# Autodesk Inventor assembly: Base
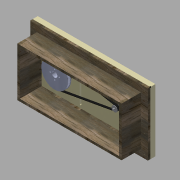
[picture p0: Inventor's stored thumbnail of the model, 180x180]
Saved by Autodesk Inventor 2019 (Build 230136000, 136)
## iProperties
Created: 2021-11-07
Part Number: Base
Document SubType Name: Assembly
Designer: Mohamed
Author: Mohamed
## Documents named in this file (11)
- F:\Semester 7\Design of mechatronics 1\SSCARA Robot\Base.iam
- F:\Semester 7\Design of mechatronics 1\SSCARA Robot\b_base_support 3.ipt
- F:\Semester 7\Design of mechatronics 1\SSCARA Robot\b_base_support 2.ipt
- F:\Semester 7\Design of mechatronics 1\SSCARA Robot\b_Base_support 1.ipt
- F:\Semester 7\Design of mechatronics 1\SSCARA Robot\thrust bearing_40mm.iam
- F:\Semester 7\Design of mechatronics 1\SSCARA Robot\b_base_cover_1.ipt
- F:\Semester 7\Design of mechatronics 1\SSCARA Robot\110 teeth gt2 pulley.ipt
- F:\Semester 7\Design of mechatronics 1\SSCARA Robot\nema 17 motor.ipt
- F:\Semester 7\Design of mechatronics 1\SSCARA Robot\ball bearing 35mm.ipt
- F:\Semester 7\Design of mechatronics 1\SSCARA Robot\GT2 pulley 20 teeth.ipt
- F:\Semester 7\Design of mechatronics 1\SSCARA Robot\belt_460mm.ipt
## Components (13 placed, 10 different names)
1. b_base_support 3:1 — Mate:4, Flush:1, Flush:2
2. b_base_support 2:1 — Mate:6, Flush:5, Flush:6
3. b_Base_support 1:1 — Mate:1, Mate:2, Mate:3, Mate:4, Flush:1, Mate:5, Flush:3, Mate:6, Flush:6, Mate:19, Flush:8, Flush:9
4. b_base_support 3:2 — Mate:5, Flush:3, Flush:4, Flush:5
5. b_base_support 2:2 — Mate:1, Mate:2, Mate:3, Flush:2, Flush:4
6. thrust bearing_40mm:1 [sub-assembly] — Mate:7, Mate:8, Mate:12
7. thrust bearing_40mm:2 [sub-assembly] — Mate:13, Mate:14
8. b_base_cover_1:1 — Mate:9, Mate:10, Mate:12, Mate:13, Mate:15, Mate:16, Mate:17, Mate:19, Flush:8, Flush:9
9. 110 teeth gt2 pulley:1 — Mate:7, Mate:8, Mate:11, Mate:14, Flush:7, Mate:21
10. nema 17 motor:1 — Mate:15, Mate:16, Mate:17, Mate:18
11. ball bearing 35mm:1 — Mate:9, Mate:10, Mate:11
12. GT2 pulley 20 teeth:1 — Mate:18, Flush:7, Mate:20, Mate:22
13. belt_460mm:1 — Mate:20, Mate:21, Mate:22
## Relationships (31: Mate 22, Flush 9)
- Mate:1: b_Base_support 1:1 ↔ b_base_support 2:2
- Mate:2: b_Base_support 1:1 ↔ b_base_support 2:2
- Mate:3: b_Base_support 1:1 ↔ b_base_support 2:2
- Mate:4: b_base_support 3:1 ↔ b_Base_support 1:1
- Flush:1: b_base_support 3:1 ↔ b_Base_support 1:1
- Flush:2: b_base_support 3:1 ↔ b_base_support 2:2
- Mate:5: b_Base_support 1:1 ↔ b_base_support 3:2
- Flush:3: b_Base_support 1:1 ↔ b_base_support 3:2
- Flush:4: b_base_support 3:2 ↔ b_base_support 2:2
- Mate:6: b_base_support 2:1 ↔ b_Base_support 1:1
- Flush:5: b_base_support 2:1 ↔ b_base_support 3:2
- Flush:6: b_base_support 2:1 ↔ b_Base_support 1:1
- Mate:7: thrust bearing_40mm:1 ↔ 110 teeth gt2 pulley:1
- Mate:8: thrust bearing_40mm:1 ↔ 110 teeth gt2 pulley:1
- Mate:9: b_base_cover_1:1 ↔ ball bearing 35mm:1
- Mate:10: b_base_cover_1:1 ↔ ball bearing 35mm:1
- Mate:11: 110 teeth gt2 pulley:1 ↔ ball bearing 35mm:1
- Mate:12: thrust bearing_40mm:1 ↔ b_base_cover_1:1
- Mate:13: thrust bearing_40mm:2 ↔ b_base_cover_1:1
- Mate:14: thrust bearing_40mm:2 ↔ 110 teeth gt2 pulley:1
- Mate:15: b_base_cover_1:1 ↔ nema 17 motor:1
- Mate:16: b_base_cover_1:1 ↔ nema 17 motor:1
- Mate:17: b_base_cover_1:1 ↔ nema 17 motor:1
- Mate:18: nema 17 motor:1 ↔ GT2 pulley 20 teeth:1
- Flush:7: 110 teeth gt2 pulley:1 ↔ GT2 pulley 20 teeth:1
- Mate:19: b_Base_support 1:1 ↔ b_base_cover_1:1
- Flush:8: b_Base_support 1:1 ↔ b_base_cover_1:1
- Flush:9: b_Base_support 1:1 ↔ b_base_cover_1:1
- Mate:20: GT2 pulley 20 teeth:1 ↔ belt_460mm:1
- Mate:21: 110 teeth gt2 pulley:1 ↔ belt_460mm:1
- Mate:22: GT2 pulley 20 teeth:1 ↔ belt_460mm:1
